# Autodesk Inventor assembly: CarPlane
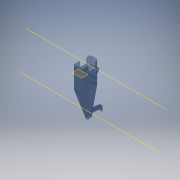
[picture p0: Inventor's stored thumbnail of the model, 180x180]
Saved by Autodesk Inventor 2017 (Build 210142000, 142)
## iProperties
Created: 2017-08-04
Part Number: CarPlane
Document SubType Name: Assembly
Designer: vmiguel
Author: vmiguel
## Documents named in this file (3)
- C:\Users\vmiguel\Dropbox\CarPlane\CarPlane.iam
- C:\Users\vmiguel\Dropbox\CarPlane\MetricsTop.ipt
- C:\Users\vmiguel\Dropbox\CarPlane\Fuselage.ipt
## Components (2 placed, 2 different names)
1. MetricsTop:1 — Flush:1, Flush:2, Flush:3, Flush:4
2. Fuselage:1 — Flush:1, Flush:2, Flush:3, Flush:4
## Relationships (4: Flush 4)
- Flush:1: MetricsTop:1 ↔ Fuselage:1
- Flush:2: MetricsTop:1 ↔ Fuselage:1
- Flush:3: MetricsTop:1 ↔ Fuselage:1
- Flush:4: MetricsTop:1 ↔ Fuselage:1
